# Autodesk Inventor assembly: main body 2
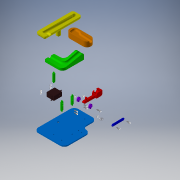
[picture p0: Inventor's stored thumbnail of the model, 180x180]
Saved by Autodesk Inventor 2016 (Build 200138000, 138)
## iProperties
Created: 2018-05-12
Part Number: main body 2
Material: 一般
Document SubType Name: Assembly
Designer: 黃胤瑋
Author: 黃胤瑋
## Documents named in this file (16)
- C:\Users\黃胤瑋\Desktop\mechanism\second generation\main body 2.iam
- C:\Users\黃胤瑋\Desktop\mechanism\second generation\馬達.ipt
- C:\Users\黃胤瑋\Desktop\mechanism\second generation\實體1.ipt
- C:\Users\黃胤瑋\Desktop\mechanism\second generation\實體2.ipt
- C:\Users\黃胤瑋\Desktop\mechanism\second generation\實體3.ipt
- C:\Users\黃胤瑋\Desktop\mechanism\second generation\實體4.ipt
- C:\Users\黃胤瑋\Desktop\mechanism\second generation\實體5.ipt
- C:\Users\黃胤瑋\Desktop\mechanism\second generation\實體7.ipt
- C:\Users\黃胤瑋\Desktop\mechanism\second generation\實體8.ipt
- C:\Users\黃胤瑋\Desktop\mechanism\second generation\實體9.ipt
- C:\Users\黃胤瑋\Desktop\mechanism\second generation\實體10.ipt
- C:\Users\黃胤瑋\Desktop\mechanism\second generation\02連桿25.ipt
- C:\Users\黃胤瑋\Desktop\mechanism\second generation\03連桿15.ipt
- C:\Users\黃胤瑋\Desktop\mechanism\second generation\JIS B 1176 - M4 x 12.ipt
- C:\Users\黃胤瑋\Desktop\mechanism\second generation\JIS B 1176 - M4 x 16.ipt
- C:\Users\黃胤瑋\Desktop\mechanism\second generation\JIS B 1181 - B M4.ipt
## Components (27 placed, 15 different names)
1. 馬達:1 — 角度:4, 齊平:2, 貼合:55, 貼合:56, 貼合:57, 貼合:58, 貼合:59, 貼合:60, 貼合:66, 角度:7
2. 實體1:1 — 貼合:3, 貼合:4, 貼合:6, 貼合:8, 角度:1, 角度:2, 貼合:12, 貼合:13, 角度:3, 角度:4, 貼合:19, 貼合:20, 角度:5, 貼合:23, 貼合:24, 角度:6, 貼合:25, 貼合:26, 貼合:27, 貼合:63
3. 實體2:1 — 貼合:3, 齊平:4, 齊平:5, 貼合:63, 貼合:64
4. 實體3:1 — 貼合:25, 貼合:26, 貼合:27
5. 實體4:1 — 貼合:21, 貼合:22, 角度:5
6. 實體5:1 — 貼合:6, 貼合:8, 角度:2, 貼合:28, 貼合:29, 貼合:30, 貼合:31, 貼合:55, 貼合:56
7. 實體7:1 — 貼合:4, 角度:1, 貼合:40, 齊平:3, 貼合:62, 齊平:5, 貼合:65
8. 實體8:1 — 貼合:19, 貼合:20, 貼合:21, 貼合:22
9. 實體9:1 — 貼合:23, 貼合:24, 角度:6
10. 實體10:1 — 貼合:48, 貼合:61, 貼合:62, 貼合:64, 貼合:65
11. 02連桿25:1 — 貼合:16, 貼合:17, 貼合:36, 貼合:37, 貼合:38, 貼合:39, 貼合:61
12. 03連桿15:1 — 齊平:2, 貼合:16, 貼合:17, 貼合:49, 貼合:66, 角度:7
13. 實體5:2 — 貼合:12, 貼合:13, 角度:3, 貼合:32, 貼合:33, 貼合:34, 貼合:35
14. JIS B 1176 - 公制 M4 x 12:1 — 貼合:28, 貼合:29, 貼合:42
15. JIS B 1176 - 公制 M4 x 16:1 — 貼合:40, 齊平:3, 貼合:43
16. JIS B 1181 (無倒角) - 公制 B M4:1 — 貼合:42, 貼合:57
17. JIS B 1176 - 公制 M4 x 12:2 — 貼合:30, 貼合:31, 貼合:45
18. JIS B 1176 - 公制 M4 x 12:3 — 貼合:32, 貼合:34, 貼合:41
19. JIS B 1176 - 公制 M4 x 12:4 — 貼合:33, 貼合:35, 貼合:44
20. JIS B 1176 - 公制 M4 x 12:5 — 貼合:36, 貼合:37, 貼合:46
21. JIS B 1176 - 公制 M4 x 12:8 — 貼合:38, 貼合:39, 貼合:47
22. JIS B 1181 (無倒角) - 公制 B M4:2 — 貼合:41, 貼合:59
23. JIS B 1181 (無倒角) - 公制 B M4:3 — 貼合:43, 齊平:4
24. JIS B 1181 (無倒角) - 公制 B M4:4 — 貼合:44, 貼合:60
25. JIS B 1181 (無倒角) - 公制 B M4:5 — 貼合:45, 貼合:58
26. JIS B 1181 (無倒角) - 公制 B M4:6 — 貼合:46, 貼合:49
27. JIS B 1181 (無倒角) - 公制 B M4:7 — 貼合:47, 貼合:48
## Relationships (62: Mate 51, Angle 7, Flush 4)
- 貼合:3 [Mate] (130 mm): 實體1:1 ↔ 實體2:1
- 貼合:4 [Mate] (130 mm): 實體1:1 ↔ 實體7:1
- 貼合:6 [Mate]: 實體1:1 ↔ 實體5:1
- 貼合:8 [Mate] (130 mm): 實體1:1 ↔ 實體5:1
- 角度:1 [Angle] (0 deg): 實體1:1 ↔ 實體7:1
- 角度:2 [Angle] (0 deg): 實體1:1 ↔ 實體5:1
- 貼合:12 [Mate]: 實體1:1 ↔ 實體5:2
- 貼合:13 [Mate] (130 mm): 實體1:1 ↔ 實體5:2
- 角度:3 [Angle] (0 deg): 實體1:1 ↔ 實體5:2
- 角度:4 [Angle] (0 deg): 馬達:1 ↔ 實體1:1
- 齊平:2 [Flush] (-200 mm): 馬達:1 ↔ 03連桿15:1
- 貼合:16 [Mate]: 02連桿25:1 ↔ 03連桿15:1
- 貼合:17 [Mate] (50 mm): 02連桿25:1 ↔ 03連桿15:1
- 貼合:19 [Mate]: 實體1:1 ↔ 實體8:1
- 貼合:20 [Mate] (230 mm): 實體1:1 ↔ 實體8:1
- 貼合:21 [Mate]: 實體4:1 ↔ 實體8:1
- 貼合:22 [Mate] (50 mm): 實體4:1 ↔ 實體8:1
- 角度:5 [Angle] (0 deg): 實體1:1 ↔ 實體4:1
- 貼合:23 [Mate]: 實體1:1 ↔ 實體9:1
- 貼合:24 [Mate] (380 mm): 實體1:1 ↔ 實體9:1
- 角度:6 [Angle] (0 deg): 實體1:1 ↔ 實體9:1
- 貼合:25 [Mate]: 實體1:1 ↔ 實體3:1
- 貼合:26 [Mate]: 實體1:1 ↔ 實體3:1
- 貼合:27 [Mate] (330 mm): 實體1:1 ↔ 實體3:1
- 貼合:28 [Mate]: 實體5:1 ↔ JIS B 1176 - 公制 M4 x 12:1
- 貼合:29 [Mate] (70 mm): 實體5:1 ↔ JIS B 1176 - 公制 M4 x 12:1
- 貼合:30 [Mate]: 實體5:1 ↔ JIS B 1176 - 公制 M4 x 12:2
- 貼合:31 [Mate] (70 mm): 實體5:1 ↔ JIS B 1176 - 公制 M4 x 12:2
- 貼合:32 [Mate]: 實體5:2 ↔ JIS B 1176 - 公制 M4 x 12:3
- 貼合:33 [Mate]: 實體5:2 ↔ JIS B 1176 - 公制 M4 x 12:4
- 貼合:34 [Mate] (70 mm): 實體5:2 ↔ JIS B 1176 - 公制 M4 x 12:3
- 貼合:35 [Mate] (70 mm): 實體5:2 ↔ JIS B 1176 - 公制 M4 x 12:4
- 貼合:36 [Mate]: 02連桿25:1 ↔ JIS B 1176 - 公制 M4 x 12:5
- 貼合:37 [Mate] (30 mm): 02連桿25:1 ↔ JIS B 1176 - 公制 M4 x 12:5
- 貼合:38 [Mate]: 02連桿25:1 ↔ JIS B 1176 - 公制 M4 x 12:8
- 貼合:39 [Mate] (30 mm): 02連桿25:1 ↔ JIS B 1176 - 公制 M4 x 12:8
- 貼合:40 [Mate]: 實體7:1 ↔ JIS B 1176 - 公制 M4 x 16:1
- 齊平:3 [Flush] (50 mm): 實體7:1 ↔ JIS B 1176 - 公制 M4 x 16:1
- 貼合:41 [Mate]: JIS B 1176 - 公制 M4 x 12:3 ↔ JIS B 1181 (無倒角) - 公制 B M4:2
- 貼合:42 [Mate]: JIS B 1176 - 公制 M4 x 12:1 ↔ JIS B 1181 (無倒角) - 公制 B M4:1
- 貼合:43 [Mate]: JIS B 1176 - 公制 M4 x 16:1 ↔ JIS B 1181 (無倒角) - 公制 B M4:3
- 貼合:44 [Mate]: JIS B 1176 - 公制 M4 x 12:4 ↔ JIS B 1181 (無倒角) - 公制 B M4:4
- 貼合:45 [Mate]: JIS B 1176 - 公制 M4 x 12:2 ↔ JIS B 1181 (無倒角) - 公制 B M4:5
- 貼合:46 [Mate]: JIS B 1176 - 公制 M4 x 12:5 ↔ JIS B 1181 (無倒角) - 公制 B M4:6
- 貼合:47 [Mate]: JIS B 1176 - 公制 M4 x 12:8 ↔ JIS B 1181 (無倒角) - 公制 B M4:7
- 貼合:48 [Mate] (10 mm): 實體10:1 ↔ JIS B 1181 (無倒角) - 公制 B M4:7
- 貼合:49 [Mate] (20 mm): 03連桿15:1 ↔ JIS B 1181 (無倒角) - 公制 B M4:6
- 齊平:4 [Flush] (20 mm): 實體2:1 ↔ JIS B 1181 (無倒角) - 公制 B M4:3
- 貼合:55 [Mate] (50 mm): 馬達:1 ↔ 實體5:1
- 貼合:56 [Mate]: 馬達:1 ↔ 實體5:1
- 貼合:57 [Mate] (50 mm): 馬達:1 ↔ JIS B 1181 (無倒角) - 公制 B M4:1
- 貼合:58 [Mate] (50 mm): 馬達:1 ↔ JIS B 1181 (無倒角) - 公制 B M4:5
- 貼合:59 [Mate] (50 mm): 馬達:1 ↔ JIS B 1181 (無倒角) - 公制 B M4:2
- 貼合:60 [Mate] (50 mm): 馬達:1 ↔ JIS B 1181 (無倒角) - 公制 B M4:4
- 貼合:61 [Mate]: 實體10:1 ↔ 02連桿25:1
- 貼合:62 [Mate]: 實體7:1 ↔ 實體10:1
- 齊平:5 [Flush]: 實體2:1 ↔ 實體7:1
- 貼合:63 [Mate]: 實體1:1 ↔ 實體2:1
- 貼合:64 [Mate] (20 mm): 實體2:1 ↔ 實體10:1
- 貼合:65 [Mate] (25 mm): 實體7:1 ↔ 實體10:1
- 貼合:66 [Mate]: 馬達:1 ↔ 03連桿15:1
- 角度:7 [Angle] (209 deg): 馬達:1 ↔ 03連桿15:1
